# Autodesk Inventor assembly: PAPER-VIEW
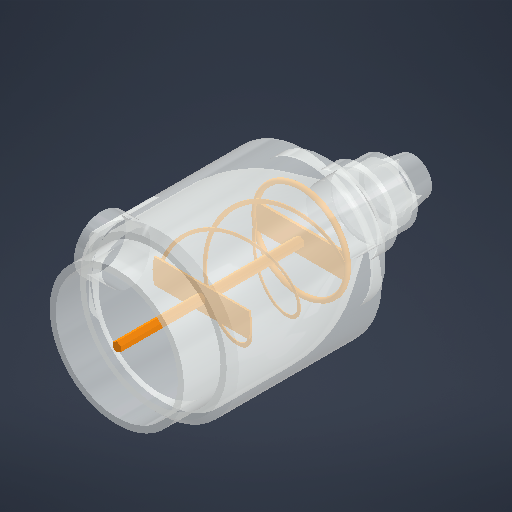
[picture p0: Inventor's stored thumbnail of the model, 512x512]
Saved by Autodesk Inventor 2025.3 (Build 293356030, 356C)
## iProperties
Created: 2025-11-12
Part Number: PAPER-VIEW
Document SubType Name: Assembly
Designer: lstk1ng
Author: lstk1ng
## Documents named in this file (4)
- C:\Users\lstk1ng\Documents\UPC\UPC-10\PROYECTO MECATRONICO 1\DISEÑO MECANICO\PAPER-VIEW.iam
- C:\Users\lstk1ng\Documents\UPC\UPC-10\PROYECTO MECATRONICO 1\DISEÑO MECANICO\COMPONENTS\MEZCLADOR-TRUPPER-80MM.ipt
- C:\Users\lstk1ng\Documents\UPC\UPC-10\PROYECTO MECATRONICO 1\DISEÑO MECANICO\LOWER-NOZZLEv2.ipt
- C:\Users\lstk1ng\Documents\UPC\UPC-10\PROYECTO MECATRONICO 1\DISEÑO MECANICO\NOZZLE-EXTRUSOR.ipt
## Components (3 placed, 3 different names)
1. MEZCLADOR-TRUPPER-80MM:1 — Mate:1, Mate:2, Mate:3
2. LOWER-NOZZLEv2:1 — Insert:1, Mate:1, Mate:2, Mate:3
3. NOZZLE-EXTRUSOR:1 — Insert:1
## Relationships (4: Mate 3, Insert 1)
- Insert:1: LOWER-NOZZLEv2:1 ↔ NOZZLE-EXTRUSOR:1
- Mate:1: MEZCLADOR-TRUPPER-80MM:1 ↔ LOWER-NOZZLEv2:1
- Mate:2: MEZCLADOR-TRUPPER-80MM:1 ↔ LOWER-NOZZLEv2:1
- Mate:3: MEZCLADOR-TRUPPER-80MM:1 ↔ LOWER-NOZZLEv2:1
